# Autodesk Inventor assembly: Złożenie ramienia robota
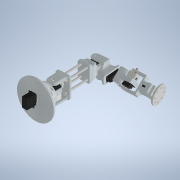
[picture p0: Inventor's stored thumbnail of the model, 180x180]
Saved by Autodesk Inventor 2021 (Build 250183000, 183)
## iProperties
Created: 2021-11-03
Part Number: Złożenie ramienia robota
Document SubType Name: Assembly
Designer: Łukasz
Author: Łukasz
## Documents named in this file (22)
- E:\GITHUB_Czołg\Szybki-Czolg-antyRadziecki\Ramie robota\Ramie robota\Złożenie ramienia robota.iam
- E:\GITHUB_Czołg\Szybki-Czolg-antyRadziecki\Ramie robota\Ramie robota\Podstawa 01-1.ipt
- E:\GITHUB_Czołg\Szybki-Czolg-antyRadziecki\Ramie robota\Ramie robota\Podstawa 01-2.ipt
- E:\GITHUB_Czołg\Szybki-Czolg-antyRadziecki\Ramie robota\Ramie robota\serwo 30x70.ipt
- E:\GITHUB_Czołg\Szybki-Czolg-antyRadziecki\Ramie robota\Ramie robota\mocowanie lozyska 10-1.ipt
- C:\Users\Łukasz\Documents\Inventor\Content Center Files\R2021\en-US\BS 292 (I)\BS 292 Part 1 - 608 - 8 x 22 x 7.ipt
- E:\GITHUB_Czołg\Szybki-Czolg-antyRadziecki\Ramie robota\Ramie robota\orczyk serwa okrągły 02-1.ipt
- E:\GITHUB_Czołg\Szybki-Czolg-antyRadziecki\Ramie robota\Ramie robota\ramie 03-1.ipt
- C:\Users\Łukasz\Documents\Inventor\Content Center Files\R2021\en-US\AS 1427(02)\AS 1427 - M8 x 16(2).ipt
- E:\GITHUB_Czołg\Szybki-Czolg-antyRadziecki\Ramie robota\Ramie robota\pręt 04-1.ipt
- E:\GITHUB_Czołg\Szybki-Czolg-antyRadziecki\Ramie robota\Ramie robota\podstawa 01-3.ipt
- E:\GITHUB_Czołg\Szybki-Czolg-antyRadziecki\Ramie robota\Ramie robota\servo 20x40.ipt
- E:\GITHUB_Czołg\Szybki-Czolg-antyRadziecki\Ramie robota\Ramie robota\ramie 03-2.ipt
- E:\GITHUB_Czołg\Szybki-Czolg-antyRadziecki\Ramie robota\Ramie robota\ramie 03-3.ipt
- E:\GITHUB_Czołg\Szybki-Czolg-antyRadziecki\Ramie robota\Ramie robota\mocowanie lozyska 10-2.ipt
- E:\GITHUB_Czołg\Szybki-Czolg-antyRadziecki\Ramie robota\Ramie robota\orczyk serwa okrągły 02-2.ipt
- E:\GITHUB_Czołg\Szybki-Czolg-antyRadziecki\Ramie robota\Ramie robota\ramie 03-4.ipt
- E:\GITHUB_Czołg\Szybki-Czolg-antyRadziecki\Ramie robota\Ramie robota\ramie03-5.ipt
- E:\GITHUB_Czołg\Szybki-Czolg-antyRadziecki\Ramie robota\Ramie robota\ramie 03-6.ipt
- E:\GITHUB_Czołg\Szybki-Czolg-antyRadziecki\Ramie robota\Ramie robota\ramie03-7.ipt
- E:\GITHUB_Czołg\Szybki-Czolg-antyRadziecki\Ramie robota\Ramie robota\mocowanie lozyska 10-3.ipt
- E:\GITHUB_Czołg\Szybki-Czolg-antyRadziecki\Ramie robota\Ramie robota\kiść.ipt
## Components (39 placed, 21 different names)
1. Podstawa 01-1:1 — Mate:1, Mate:2, Mate:3
2. Podstawa 01-2:1 — Mate:4, Mate:5, Mate:6, Rigid:5
3. serwo 30x70:1 — Mate:1, Mate:2, Mate:3, Mate:4, Mate:5, Mate:6, Mate:7, Flush:2, Rotational:19, Mate:8, Mate:9, Mate:10, Mate:11
4. mocowanie lozyska 10-1:1 — Mate:7, Flush:2, Rigid:14, Mate:8
5. BS 292: Part 1 (I) (Metric) 608 - 8 x 22 x 7:1 — Rigid:14, Rigid:10
6. orczyk serwa okrągły 02-1:1 — Rotational:19, Rigid:13
7. ramie 03-1:1 — Rigid:1, Rigid:2, Rigid:3, Rigid:4, Rigid:13, Rigid:12
8. AS 1427 - Metric M8 x 16:1 — Rigid:12
9. pręt 04-1:1 — Rigid:1, Rotational:11
10. pręt 04-1:2 — Rigid:2, Rotational:12
11. pręt 04-1:3 — Rigid:3
12. pręt 04-1:4 — Rigid:4
13. podstawa 01-3:1 — Mate:9, Mate:10, Mate:11
14. servo 20x40:1 — Mate:12, Mate:13, Mate:14, Mate:15, Mate:16, Mate:17, Mate:18, Rotational:22
15. ramie 03-2:1 — Mate:12, Mate:13, Mate:14, Flush:3, Flush:4, Rotational:11, Rotational:12
16. ramie 03-3:1 — Mate:15, Flush:3, Flush:4
17. mocowanie lozyska 10-2:1 — Mate:16, Mate:17, Mate:18, Rigid:20
18. orczyk serwa okrągły 02-2:1 — Rotational:22, Rigid:15
19. BS 292: Part 1 (I) (Metric) 608 - 8 x 22 x 7:2 — Rigid:20
20. ramie 03-4:1 — Mate:19, Mate:20, Mate:21, Rigid:15, Flush:5, Flush:6, Rigid:8
21. servo 20x40:2 — Mate:19, Mate:20, Mate:21, Mate:22, Rotational:23
22. ramie03-5:1 — Mate:22, Flush:5, Flush:6
23. orczyk serwa okrągły 02-2:2 — Rotational:23, Rigid:19
24. ramie 03-6:1 — Rigid:19, Mate:23, Mate:24, Mate:25, Mate:26, Flush:7, Flush:8
25. servo 20x40:3 — Mate:23, Mate:24, Mate:25, Mate:27, Mate:28, Mate:29, Rotational:24
26. ramie 03-3:2 — Mate:26, Flush:7, Flush:8
27. orczyk serwa okrągły 02-2:3 — Rigid:5, Rigid:21
28. servo 20x40:4 — Rigid:21
29. mocowanie lozyska 10-2:2 — Mate:27, Mate:28, Mate:29, Rigid:6
30. orczyk serwa okrągły 02-2:4 — Rigid:18, Rotational:24
31. ramie 03-4:2 — Rigid:18, Rigid:9, Mate:30, Mate:31, Mate:32, Mate:33, Flush:9, Flush:10
32. BS 292: Part 1 (I) (Metric) 608 - 8 x 22 x 7:3 — Rigid:6
33. AS 1427 - Metric M8 x 16:2 — Rigid:8
34. AS 1427 - Metric M8 x 16:3 — Rigid:9
35. servo 20x40:5 — Mate:30, Mate:31, Mate:32, Rigid:11
36. ramie03-7:1 — Mate:33, Flush:9, Flush:10
37. mocowanie lozyska 10-3:1 — Rigid:10
38. orczyk serwa okrągły 02-2:5 — Rigid:11, Rigid:22
39. kiść:1 — Rigid:22
## Relationships (67: Mate 33, WeldJoint 19, Flush 9, RevoluteJoint 6)
- Mate:1: Podstawa 01-1:1 ↔ serwo 30x70:1
- Mate:2: Podstawa 01-1:1 ↔ serwo 30x70:1
- Mate:3: Podstawa 01-1:1 ↔ serwo 30x70:1
- Mate:4: Podstawa 01-2:1 ↔ serwo 30x70:1
- Mate:5: Podstawa 01-2:1 ↔ serwo 30x70:1
- Mate:6: Podstawa 01-2:1 ↔ serwo 30x70:1
- Mate:7: serwo 30x70:1 ↔ mocowanie lozyska 10-1:1
- Flush:2: serwo 30x70:1 ↔ mocowanie lozyska 10-1:1
- Rigid:14 [WeldJoint]: mocowanie lozyska 10-1:1 ↔ BS 292: Part 1 (I) (Metric) 608 - 8 x 22 x 7:1
- Rotational:19 [RevoluteJoint]: serwo 30x70:1 ↔ orczyk serwa okrągły 02-1:1
- Mate:8: serwo 30x70:1 ↔ mocowanie lozyska 10-1:1
- Rigid:1 [WeldJoint] (5 mm): ramie 03-1:1 ↔ pręt 04-1:1
- Rigid:2 [WeldJoint] (5 mm): ramie 03-1:1 ↔ pręt 04-1:2
- Rigid:3 [WeldJoint] (5 mm): ramie 03-1:1 ↔ pręt 04-1:3
- Rigid:4 [WeldJoint] (5 mm): ramie 03-1:1 ↔ pręt 04-1:4
- Mate:9: serwo 30x70:1 ↔ podstawa 01-3:1
- Mate:10: serwo 30x70:1 ↔ podstawa 01-3:1
- Mate:11: serwo 30x70:1 ↔ podstawa 01-3:1
- Mate:12: servo 20x40:1 ↔ ramie 03-2:1
- Mate:13: servo 20x40:1 ↔ ramie 03-2:1
- Mate:14: servo 20x40:1 ↔ ramie 03-2:1
- Mate:15: servo 20x40:1 ↔ ramie 03-3:1
- Flush:3: ramie 03-2:1 ↔ ramie 03-3:1
- Flush:4: ramie 03-2:1 ↔ ramie 03-3:1
- Mate:16: servo 20x40:1 ↔ mocowanie lozyska 10-2:1
- Mate:17: servo 20x40:1 ↔ mocowanie lozyska 10-2:1
- Mate:18: servo 20x40:1 ↔ mocowanie lozyska 10-2:1
- Rotational:22 [RevoluteJoint]: servo 20x40:1 ↔ orczyk serwa okrągły 02-2:1
- Rigid:20 [WeldJoint]: mocowanie lozyska 10-2:1 ↔ BS 292: Part 1 (I) (Metric) 608 - 8 x 22 x 7:2
- Rigid:13 [WeldJoint]: orczyk serwa okrągły 02-1:1 ↔ ramie 03-1:1
- Rigid:12 [WeldJoint]: ramie 03-1:1 ↔ AS 1427 - Metric M8 x 16:1
- Rotational:11 [RevoluteJoint]: pręt 04-1:1 ↔ ramie 03-2:1
- Rotational:12 [RevoluteJoint]: pręt 04-1:2 ↔ ramie 03-2:1
- Mate:19: ramie 03-4:1 ↔ servo 20x40:2
- Mate:20: ramie 03-4:1 ↔ servo 20x40:2
- Mate:21: ramie 03-4:1 ↔ servo 20x40:2
- Rigid:15 [WeldJoint]: orczyk serwa okrągły 02-2:1 ↔ ramie 03-4:1
- Mate:22: servo 20x40:2 ↔ ramie03-5:1
- Flush:5: ramie 03-4:1 ↔ ramie03-5:1
- Flush:6: ramie 03-4:1 ↔ ramie03-5:1
- Rotational:23 [RevoluteJoint]: servo 20x40:2 ↔ orczyk serwa okrągły 02-2:2
- Rigid:19 [WeldJoint]: orczyk serwa okrągły 02-2:2 ↔ ramie 03-6:1
- Mate:23: ramie 03-6:1 ↔ servo 20x40:3
- Mate:24: ramie 03-6:1 ↔ servo 20x40:3
- Mate:25: ramie 03-6:1 ↔ servo 20x40:3
- Mate:26: ramie 03-6:1 ↔ ramie 03-3:2
- Flush:7: ramie 03-6:1 ↔ ramie 03-3:2
- Flush:8: ramie 03-6:1 ↔ ramie 03-3:2
- Rigid:5 [WeldJoint]: Podstawa 01-2:1 ↔ orczyk serwa okrągły 02-2:3
- Rigid:21 [WeldJoint]: orczyk serwa okrągły 02-2:3 ↔ servo 20x40:4
- Mate:27: servo 20x40:3 ↔ mocowanie lozyska 10-2:2
- Mate:28: servo 20x40:3 ↔ mocowanie lozyska 10-2:2
- Mate:29: servo 20x40:3 ↔ mocowanie lozyska 10-2:2
- Rigid:6 [WeldJoint]: mocowanie lozyska 10-2:2 ↔ BS 292: Part 1 (I) (Metric) 608 - 8 x 22 x 7:3
- Rigid:18 [WeldJoint]: orczyk serwa okrągły 02-2:4 ↔ ramie 03-4:2
- Rigid:8 [WeldJoint]: ramie 03-4:1 ↔ AS 1427 - Metric M8 x 16:2
- Rigid:9 [WeldJoint]: ramie 03-4:2 ↔ AS 1427 - Metric M8 x 16:3
- Mate:30: ramie 03-4:2 ↔ servo 20x40:5
- Mate:31: ramie 03-4:2 ↔ servo 20x40:5
- Mate:32: ramie 03-4:2 ↔ servo 20x40:5
- Mate:33: ramie 03-4:2 ↔ ramie03-7:1
- Flush:9: ramie 03-4:2 ↔ ramie03-7:1
- Flush:10: ramie 03-4:2 ↔ ramie03-7:1
- Rigid:10 [WeldJoint]: BS 292: Part 1 (I) (Metric) 608 - 8 x 22 x 7:1 ↔ mocowanie lozyska 10-3:1
- Rigid:11 [WeldJoint]: servo 20x40:5 ↔ orczyk serwa okrągły 02-2:5
- Rigid:22 [WeldJoint]: orczyk serwa okrągły 02-2:5 ↔ kiść:1
- Rotational:24 [RevoluteJoint]: servo 20x40:3 ↔ orczyk serwa okrągły 02-2:4
